# Autodesk Inventor assembly: Bouton
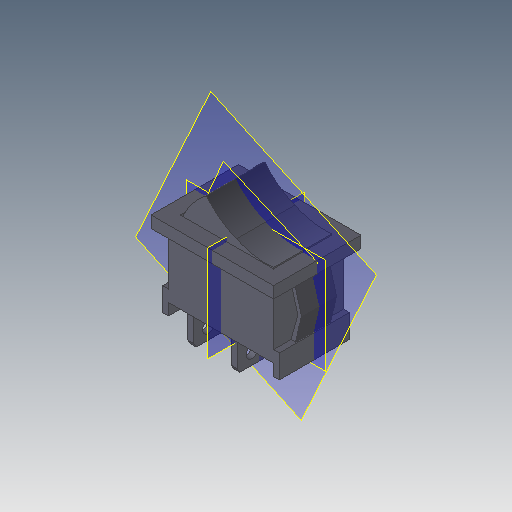
[picture p0: Inventor's stored thumbnail of the model, 512x512]
Saved by Autodesk Inventor 2017 (Build 210142000, 142)
## iProperties
Created: 2016-05-14
Part Number: Bouton
Document SubType Name: Assembly
Project: 1420 Vauban 3D XL
Stock Number: 1420-09-03
## Documents named in this file (6)
- W:\Professionnel\Conception FABLAB\1420-Vauban 3D XL\1420-09 Connectique\1420-09-10 Bouton\1420-09-03 Bouton.iam
- W:\Professionnel\Conception FABLAB\1420-Vauban 3D XL\1420-09 Connectique\1420-09-10 Bouton\Polo2.ipt
- W:\Professionnel\Conception FABLAB\1420-Vauban 3D XL\1420-09 Connectique\1420-09-10 Bouton\Pieza2.ipt
- W:\Professionnel\Conception FABLAB\1420-Vauban 3D XL\1420-09 Connectique\1420-09-10 Bouton\Sw.ipt
- W:\Professionnel\Conception FABLAB\1420-Vauban 3D XL\1420-09 Connectique\1420-09-10 Bouton\InteriorSw.ipt
- W:\Professionnel\Conception FABLAB\1420-Vauban 3D XL\1420-09 Connectique\1420-09-10 Bouton\Base.ipt
## Components (5 placed, 5 different names)
1. Base:1 — Nivelación:1, Nivelación:2, Coincidencia:1, Coincidencia:2, Simetría:1, Affleurement:6, Affleurement:7, Affleurement:8
2. Polo2:1 — Nivelación:1, Nivelación:4, Nivelación:5
3. Pieza2:1 — Nivelación:2
4. Sw:1 — Coincidencia:1, Coincidencia:2, Simetría:1, Tangente:1
5. InteriorSw:1 — Nivelación:4, Tangente:1, Nivelación:5
## Relationships (11: Flush 7, Mate 2, Symmetry 1, Tangent 1)
- Nivelación:1 [Flush]: Base:1 ↔ Polo2:1
- Nivelación:2 [Flush]: Base:1 ↔ Pieza2:1
- Coincidencia:1 [Mate]: Base:1 ↔ Sw:1
- Coincidencia:2 [Mate]: Base:1 ↔ Sw:1
- Simetría:1 [Symmetry]: Base:1 ↔ Sw:1
- Nivelación:4 [Flush]: Polo2:1 ↔ InteriorSw:1
- Tangente:1 (-2 mm): Sw:1 ↔ InteriorSw:1
- Nivelación:5 [Flush] (1 mm): Polo2:1 ↔ InteriorSw:1
- Affleurement:6 [Flush] (-10 mm): Base:1
- Affleurement:7 [Flush] (-6 mm): Base:1
- Affleurement:8 [Flush] (-10 mm): Base:1
